# Autodesk Inventor assembly: WheelAssemblyWFrame
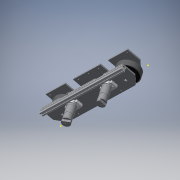
[picture p0: Inventor's stored thumbnail of the model, 180x180]
Saved by Autodesk Inventor 2016 (Build 200138000, 138)
## iProperties
Created: 2016-10-08
Part Number: WheelAssemblyWFrame
Document SubType Name: Assembly
Designer: RoboticsUser
Author: RoboticsUser
## Documents named in this file (4)
- C:\Robotics\2016-17_CAD\WheelAssemblyWFrame.iam
- C:\Robotics\2016-17_CAD\WheelAssembly.iam
- C:\Robotics\CAD\2015-16\COTSParts\Bosch Extrusion\Bosch 20x20.ipt
- C:\Robotics\CAD\2015-16\COTSParts\Bosch Extrusion\6mm block nut M4.ipt
## Components (7 placed, 3 different names)
1. WheelAssembly:2 [sub-assembly] — Flush:2, Insert:1, Insert:2, Insert:3, Insert:4, Insert:5
2. Bosch 20x20:1 — Flush:2, Mate:1, Mate:2
3. 6mm block nut M4:6 — Insert:1, Mate:1, Mate:2
4. 6mm block nut M4:7 — Insert:2
5. 6mm block nut M4:8 — Insert:4
6. 6mm block nut M4:9 — Insert:5
7. 6mm block nut M4:10 — Insert:3
## Relationships (8: Insert 5, Mate 2, Flush 1)
- Flush:2: WheelAssembly:2 ↔ Bosch 20x20:1
- Insert:1: WheelAssembly:2 ↔ 6mm block nut M4:6
- Insert:2: WheelAssembly:2 ↔ 6mm block nut M4:7
- Insert:3: WheelAssembly:2 ↔ 6mm block nut M4:10
- Insert:4: WheelAssembly:2 ↔ 6mm block nut M4:8
- Insert:5: WheelAssembly:2 ↔ 6mm block nut M4:9
- Mate:1: Bosch 20x20:1 ↔ 6mm block nut M4:6
- Mate:2: Bosch 20x20:1 ↔ 6mm block nut M4:6
